# Autodesk Inventor assembly: 1000_Coil_Positioning_Assembly_MPSv2_v4
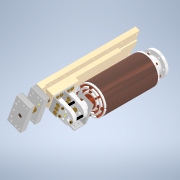
[picture p0: Inventor's stored thumbnail of the model, 180x180]
Saved by Autodesk Inventor 2021 (Build 250183000, 183)
## iProperties
Created: 2020-11-12
Part Number: 1000_Coil_Positioning_Assembly_MPSv2_v4
Document SubType Name: Assembly
Designer: Admin
Author: Admin
## Documents named in this file (23)
- C:\Users\Barksdale\Dropbox (MIT)\MPI Group Folder\MPS\MPSV2\1xxx Assemblies\1000_Coil_Positioning_Assembly_MPSv2_v4.iam
- C:\Users\Barksdale\Dropbox (MIT)\MPI Group Folder\MPS\MPSV2\2xxx Coil Formers and Parts\20xx Rx Coil\200x Rx Coil Solenoid Former\2000_Rx_Coil_Former_MPSv2_v2.ipt
- C:\Users\Barksdale\Dropbox (MIT)\MPI Group Folder\MPS\MPSV2\2xxx Coil Formers and Parts\20xx Rx Coil\200x Rx Coil Solenoid Former\2001_Fiberglass_Rod_MPSv2_v1.ipt
- C:\Users\Barksdale\Dropbox (MIT)\MPI Group Folder\MPS\MPSV2\2xxx Coil Formers and Parts\21xx Tx Coil\210x Tx Coil Solenoid Former\2100_Tx_Coil_Former_MPSv2_v3.ipt
- C:\Users\Barksdale\Dropbox (MIT)\MPI Group Folder\MPS\MPSV2\McMaster Carr Parts\94995A470_BRONZE THREADED ROD.ipt
- C:\Users\Barksdale\Dropbox (MIT)\MPI Group Folder\MPS\MPSV2\3xxx Coil Positioning and Support\30xx_Tx_Rx_Relative_Positioning\3004_Brass_Nut_0.25_20_Tx_Rx_Relative_Positioning_MPSv2_v1.ipt
- C:\Users\Barksdale\Dropbox (MIT)\MPI Group Folder\MPS\MPSV2\McMaster Carr Parts\98813A033_BRASS THREADED ROD.ipt
- C:\Users\Barksdale\Dropbox (MIT)\MPI Group Folder\MPS\MPSV2\3xxx Coil Positioning and Support\31xx_Bias_Coil_Positioning\311x_Bias_Tx_Rx_Relative_Positioning\3114_Brass_Nut_0.5_20_Tx_Rx_Relative_Positioning_MPSv2_v1.ipt
- C:\Users\Barksdale\Dropbox (MIT)\MPI Group Folder\MPS\MPSV2\McMaster Carr Parts\2705T140_LIGHT DUTY DRY-RUNNING FLANGED SLEEVE BEARING.ipt
- C:\Users\Barksdale\Dropbox (MIT)\MPI Group Folder\MPS\MPSV2\McMaster Carr Parts\2705T260_LIGHT DUTY DRY-RUNNING FLANGED SLEEVE BEARING.ipt
- C:\Users\Barksdale\Dropbox (MIT)\MPI Group Folder\MPS\MPSV2\3xxx Coil Positioning and Support\31xx_Bias_Coil_Positioning\311x_Bias_Tx_Rx_Relative_Positioning\3113_Bias_TxRx_Relative_Adapter_MPSv2_v1.ipt
- C:\Users\Barksdale\Dropbox (MIT)\MPI Group Folder\MPS\MPSV2\3xxx Coil Positioning and Support\31xx_Bias_Coil_Positioning\310x_Bias_Coil_Chasis_Mounting\3101_Bias_Coil_Mounting_Flange_MPSv2_v2.ipt
- C:\Users\Barksdale\Dropbox (MIT)\MPI Group Folder\MPS\MPSV2\2xxx Coil Formers and Parts\22xx Bias Coil\4000_Cu_Bias_Shielding_(McMaster_50475K18)_MPSv2_v2.ipt
- C:\Users\Barksdale\Dropbox (MIT)\MPI Group Folder\MPS\MPSV2\3xxx Coil Positioning and Support\30xx_Tx_Rx_Relative_Positioning\3000_Tx_Rx_Relative_Position_Adjust_Tx_Adadpter_Male_MPSv2_v5.ipt
- C:\Users\Barksdale\Dropbox (MIT)\MPI Group Folder\MPS\MPSV2\3xxx Coil Positioning and Support\31xx_Bias_Coil_Positioning\311x_Bias_Tx_Rx_Relative_Positioning\3112_Bias_TxRx_Relative_Dovetail_Male_MPSv2_v3.ipt
- C:\Users\Barksdale\Dropbox (MIT)\MPI Group Folder\MPS\MPSV2\3xxx Coil Positioning and Support\30xx_Tx_Rx_Relative_Positioning\3001_Tx_Rx_Relative_Position_Adjust_Tx_Adadpter_Female_MPSv2_v4.ipt
- C:\Users\Barksdale\Dropbox (MIT)\MPI Group Folder\MPS\MPSV2\3xxx Coil Positioning and Support\31xx_Bias_Coil_Positioning\311x_Bias_Tx_Rx_Relative_Positioning\3110_Bias_TxRx_Relative_Dovetail_Mount_Bracket_MPSv2_v4.ipt
- C:\Users\Barksdale\Dropbox (MIT)\MPI Group Folder\MPS\MPSV2\3xxx Coil Positioning and Support\31xx_Bias_Coil_Positioning\311x_Bias_Tx_Rx_Relative_Positioning\3111_Bias_TxRx_Relative_Dovetail_Female_MPSv2_v4.ipt
- C:\Users\Barksdale\Dropbox (MIT)\MPI Group Folder\MPS\MPSV2\3xxx Coil Positioning and Support\30xx_Tx_Rx_Relative_Positioning\3002_92451A838_BRASS FLAT HEAD SLOTTED MACHINE SCREW.ipt
- C:\Users\Barksdale\Dropbox (MIT)\MPI Group Folder\MPS\MPSV2\3xxx Coil Positioning and Support\30xx_Tx_Rx_Relative_Positioning\3003_95130A160_BRASS NARROW HEX NUT.ipt
- C:\Users\Barksdale\Dropbox (MIT)\MPI Group Folder\MPS\MPSV2\3xxx Coil Positioning and Support\31xx_Bias_Coil_Positioning\311x_Bias_Tx_Rx_Relative_Positioning\3115_94070A550_BRASS PAN HEAD PHILLIPS MACHINE SCREW.ipt
- C:\Users\Barksdale\Dropbox (MIT)\MPI Group Folder\MPS\MPSV2\1xxx Assemblies\10xx_Coil_Positioning_Assemblies\1002_Bias_Coil_MPSv2_v3.iam
- C:\Users\Barksdale\Dropbox (MIT)\MPI Group Folder\MPS\MPSV2\3xxx Coil Positioning and Support\31xx_Bias_Coil_Positioning\310x_Bias_Coil_Chasis_Mounting\3102_Biax_Coil_Mounting_Bracket_MPSv2_v1.ipt
## Components (46 placed, 22 different names)
1. 2000_Rx_Coil_Former_MPSv2_v2:1 — Mate:6, Mate:7, Mate:9, Angle:1, Flush:4
2. 2001_Fiberglass_Rod_MPSv2_v1:1 — Mate:6, Mate:7, Mate:20, Mate:124
3. 4000_Cu_Bias_Shielding_(McMaster_50475K18)_MPSv2_v2:1 — Mate:8, Mate:10, Mate:24, Mate:119, Mate:120, Mate:175, Mate:177, Mate:178
4. 2100_Tx_Coil_Former_MPSv2_v3:1 — Mate:8, Mate:9, Mate:10, Angle:1, Mate:25, Mate:26, Flush:4
5. 94995A470_BRONZE THREADED ROD:1 — Mate:20, Mate:81, Mate:124, Mate:128
6. 3004_Brass_Nut_0.25_20_Tx_Rx_Relative_Positioning_MPSv2_v1:1 — Mate:74, Mate:75, Mate:76, Mate:77
7. 3000_Tx_Rx_Relative_Position_Adjust_Tx_Adadpter_Male_MPSv2_v5:1 — Mate:24, Mate:25, Mate:26, Mate:129, Mate:133
8. 3110_Bias_TxRx_Relative_Dovetail_Mount_Bracket_MPSv2_v4:2 — Mate:83, Mate:130, Mate:131, Mate:141, Mate:142, Mate:155, Mate:157, Mate:160, Mate:161, Mate:166, Mate:167, Mate:168, Mate:169, Mate:174
9. 3110_Bias_TxRx_Relative_Dovetail_Mount_Bracket_MPSv2_v4:1 — Mate:56, Mate:137, Mate:139, Mate:140, Mate:154, Mate:165, Mate:170, Mate:171, Mate:172, Mate:173
10. 3111_Bias_TxRx_Relative_Dovetail_Female_MPSv2_v4:1 — Mate:56, Mate:59, Mate:62, Mate:63, Mate:83, Mate:141, Mate:142, Mate:144
11. 98813A033_BRASS THREADED ROD:1 — Mate:59, Mate:64, Mate:65, Mate:144
12. 3112_Bias_TxRx_Relative_Dovetail_Male_MPSv2_v3:1 — Mate:62, Mate:63, Mate:99, Mate:100, Mate:125, Angle:2
13. 98813A033_BRASS THREADED ROD:2 — Mate:64, Mate:65, Mate:91
14. 3114_Brass_Nut_0.5_20_Tx_Rx_Relative_Positioning_MPSv2_v1:1 — Mate:87, Mate:88, Mate:89, Mate:90
15. 2705T140_LIGHT DUTY DRY-RUNNING FLANGED SLEEVE BEARING:1 — Mate:74, Mate:75, Mate:135, Mate:136
16. 2705T140_LIGHT DUTY DRY-RUNNING FLANGED SLEEVE BEARING:2 — Mate:76, Mate:77, Mate:81, Mate:134
17. 2705T260_LIGHT DUTY DRY-RUNNING FLANGED SLEEVE BEARING:1 — Mate:87, Mate:90, Mate:91, Mate:102
18. 2705T260_LIGHT DUTY DRY-RUNNING FLANGED SLEEVE BEARING:2 — Mate:88, Mate:89, Mate:98, Mate:103
19. 3113_Bias_TxRx_Relative_Adapter_MPSv2_v1:1 — Mate:99, Mate:100, Mate:102, Mate:104, Mate:105, Mate:125
20. 3113_Bias_TxRx_Relative_Adapter_MPSv2_v1:2 — Mate:98, Mate:103, Mate:104, Mate:105
21. 3101_Bias_Coil_Mounting_Flange_MPSv2_v2:1 — Mate:119, Mate:120, Mate:176
22. 1002_Bias_Coil_MPSv2_v3:1 [sub-assembly] — Mate:175, Mate:176
23. 3001_Tx_Rx_Relative_Position_Adjust_Tx_Adadpter_Female_MPSv2_v4:1 — Mate:128, Mate:129, Mate:130, Mate:131, Mate:133, Mate:134, Flush:6, Mate:145, Mate:146, Mate:147, Flush:7, Flush:8, Flush:9, Mate:155, Mate:156, Mate:158, Mate:159
24. 3001_Tx_Rx_Relative_Position_Adjust_Tx_Adadpter_Female_MPSv2_v4:2 — Mate:135, Flush:6, Mate:136, Mate:137, Mate:139, Mate:140, Mate:148, Mate:149, Mate:150, Mate:154, Mate:162, Mate:163, Mate:164
25. 3002_92451A838_BRASS FLAT HEAD SLOTTED MACHINE SCREW:1 — Mate:145, Flush:7, Mate:151
26. 3002_92451A838_BRASS FLAT HEAD SLOTTED MACHINE SCREW:2 — Mate:147, Flush:8, Mate:153
27. 3002_92451A838_BRASS FLAT HEAD SLOTTED MACHINE SCREW:3 — Mate:146, Flush:9, Mate:152
28. 3003_95130A160_BRASS NARROW HEX NUT:1 — Mate:150, Mate:152
29. 3003_95130A160_BRASS NARROW HEX NUT:2 — Mate:148, Mate:153
30. 3003_95130A160_BRASS NARROW HEX NUT:3 — Mate:149, Mate:151
31. 3115_94070A550_BRASS PAN HEAD PHILLIPS MACHINE SCREW:1 — Mate:156, Mate:157
32. 3115_94070A550_BRASS PAN HEAD PHILLIPS MACHINE SCREW:2 — Mate:159, Mate:160
33. 3115_94070A550_BRASS PAN HEAD PHILLIPS MACHINE SCREW:3 — Mate:158, Mate:161
34. 3115_94070A550_BRASS PAN HEAD PHILLIPS MACHINE SCREW:4 — Flush:10, Flush:11, Mate:162, Mate:165
35. 3115_94070A550_BRASS PAN HEAD PHILLIPS MACHINE SCREW:5 — Flush:10, Mate:163
36. 3115_94070A550_BRASS PAN HEAD PHILLIPS MACHINE SCREW:6 — Flush:11, Mate:164
37. 3115_94070A550_BRASS PAN HEAD PHILLIPS MACHINE SCREW:7 — Flush:18, Mate:166, Mate:174
38. 3115_94070A550_BRASS PAN HEAD PHILLIPS MACHINE SCREW:8 — Flush:16, Mate:168
39. 3115_94070A550_BRASS PAN HEAD PHILLIPS MACHINE SCREW:9 — Flush:17, Mate:167
40. 3115_94070A550_BRASS PAN HEAD PHILLIPS MACHINE SCREW:10 — Flush:15, Mate:169
41. 3115_94070A550_BRASS PAN HEAD PHILLIPS MACHINE SCREW:11 — Flush:12, Flush:14, Flush:15, Flush:16, Flush:17, Flush:18, Mate:170
42. 3115_94070A550_BRASS PAN HEAD PHILLIPS MACHINE SCREW:12 — Flush:12, Flush:13, Mate:172
43. 3115_94070A550_BRASS PAN HEAD PHILLIPS MACHINE SCREW:13 — Flush:13, Mate:173
44. 3115_94070A550_BRASS PAN HEAD PHILLIPS MACHINE SCREW:14 — Flush:14, Mate:171
45. 3102_Biax_Coil_Mounting_Bracket_MPSv2_v1:1 — Mate:177, Mate:178, Mate:179, Flush:19, Flush:20
46. 3110_Bias_TxRx_Relative_Dovetail_Mount_Bracket_MPSv2_v4:3 — Mate:179, Flush:19, Angle:2, Flush:20
## Relationships (104: Mate 86, Flush 16, Angle 2)
- Mate:6: 2000_Rx_Coil_Former_MPSv2_v2:1 ↔ 2001_Fiberglass_Rod_MPSv2_v1:1
- Mate:7: 2000_Rx_Coil_Former_MPSv2_v2:1 ↔ 2001_Fiberglass_Rod_MPSv2_v1:1
- Mate:8: 4000_Cu_Bias_Shielding_(McMaster_50475K18)_MPSv2_v2:1 ↔ 2100_Tx_Coil_Former_MPSv2_v3:1
- Mate:9: 2000_Rx_Coil_Former_MPSv2_v2:1 ↔ 2100_Tx_Coil_Former_MPSv2_v3:1
- Mate:10: 4000_Cu_Bias_Shielding_(McMaster_50475K18)_MPSv2_v2:1 ↔ 2100_Tx_Coil_Former_MPSv2_v3:1
- Angle:1 (0 deg): 2000_Rx_Coil_Former_MPSv2_v2:1 ↔ 2100_Tx_Coil_Former_MPSv2_v3:1
- Mate:20: 2001_Fiberglass_Rod_MPSv2_v1:1 ↔ 94995A470_BRONZE THREADED ROD:1
- Mate:24: 4000_Cu_Bias_Shielding_(McMaster_50475K18)_MPSv2_v2:1 ↔ 3000_Tx_Rx_Relative_Position_Adjust_Tx_Adadpter_Male_MPSv2_v5:1
- Mate:25: 2100_Tx_Coil_Former_MPSv2_v3:1 ↔ 3000_Tx_Rx_Relative_Position_Adjust_Tx_Adadpter_Male_MPSv2_v5:1
- Mate:26: 2100_Tx_Coil_Former_MPSv2_v3:1 ↔ 3000_Tx_Rx_Relative_Position_Adjust_Tx_Adadpter_Male_MPSv2_v5:1
- Mate:56: 3110_Bias_TxRx_Relative_Dovetail_Mount_Bracket_MPSv2_v4:1 ↔ 3111_Bias_TxRx_Relative_Dovetail_Female_MPSv2_v4:1
- Mate:59: 3111_Bias_TxRx_Relative_Dovetail_Female_MPSv2_v4:1 ↔ 98813A033_BRASS THREADED ROD:1
- Mate:62: 3111_Bias_TxRx_Relative_Dovetail_Female_MPSv2_v4:1 ↔ 3112_Bias_TxRx_Relative_Dovetail_Male_MPSv2_v3:1
- Mate:63: 3111_Bias_TxRx_Relative_Dovetail_Female_MPSv2_v4:1 ↔ 3112_Bias_TxRx_Relative_Dovetail_Male_MPSv2_v3:1
- Mate:64: 98813A033_BRASS THREADED ROD:1 ↔ 98813A033_BRASS THREADED ROD:2
- Mate:65 (-5 mm): 98813A033_BRASS THREADED ROD:1 ↔ 98813A033_BRASS THREADED ROD:2
- Mate:74: 3004_Brass_Nut_0.25_20_Tx_Rx_Relative_Positioning_MPSv2_v1:1 ↔ 2705T140_LIGHT DUTY DRY-RUNNING FLANGED SLEEVE BEARING:1
- Mate:75: 3004_Brass_Nut_0.25_20_Tx_Rx_Relative_Positioning_MPSv2_v1:1 ↔ 2705T140_LIGHT DUTY DRY-RUNNING FLANGED SLEEVE BEARING:1
- Mate:76: 3004_Brass_Nut_0.25_20_Tx_Rx_Relative_Positioning_MPSv2_v1:1 ↔ 2705T140_LIGHT DUTY DRY-RUNNING FLANGED SLEEVE BEARING:2
- Mate:77: 3004_Brass_Nut_0.25_20_Tx_Rx_Relative_Positioning_MPSv2_v1:1 ↔ 2705T140_LIGHT DUTY DRY-RUNNING FLANGED SLEEVE BEARING:2
- Mate:81: 94995A470_BRONZE THREADED ROD:1 ↔ 2705T140_LIGHT DUTY DRY-RUNNING FLANGED SLEEVE BEARING:2
- Mate:83: 3110_Bias_TxRx_Relative_Dovetail_Mount_Bracket_MPSv2_v4:2 ↔ 3111_Bias_TxRx_Relative_Dovetail_Female_MPSv2_v4:1
- Mate:87: 3114_Brass_Nut_0.5_20_Tx_Rx_Relative_Positioning_MPSv2_v1:1 ↔ 2705T260_LIGHT DUTY DRY-RUNNING FLANGED SLEEVE BEARING:1
- Mate:88: 3114_Brass_Nut_0.5_20_Tx_Rx_Relative_Positioning_MPSv2_v1:1 ↔ 2705T260_LIGHT DUTY DRY-RUNNING FLANGED SLEEVE BEARING:2
- Mate:89: 3114_Brass_Nut_0.5_20_Tx_Rx_Relative_Positioning_MPSv2_v1:1 ↔ 2705T260_LIGHT DUTY DRY-RUNNING FLANGED SLEEVE BEARING:2
- Mate:90: 3114_Brass_Nut_0.5_20_Tx_Rx_Relative_Positioning_MPSv2_v1:1 ↔ 2705T260_LIGHT DUTY DRY-RUNNING FLANGED SLEEVE BEARING:1
- Mate:91: 98813A033_BRASS THREADED ROD:2 ↔ 2705T260_LIGHT DUTY DRY-RUNNING FLANGED SLEEVE BEARING:1
- Mate:98: 2705T260_LIGHT DUTY DRY-RUNNING FLANGED SLEEVE BEARING:2 ↔ 3113_Bias_TxRx_Relative_Adapter_MPSv2_v1:2
- Mate:99: 3112_Bias_TxRx_Relative_Dovetail_Male_MPSv2_v3:1 ↔ 3113_Bias_TxRx_Relative_Adapter_MPSv2_v1:1
- Mate:100: 3112_Bias_TxRx_Relative_Dovetail_Male_MPSv2_v3:1 ↔ 3113_Bias_TxRx_Relative_Adapter_MPSv2_v1:1
- Mate:102: 2705T260_LIGHT DUTY DRY-RUNNING FLANGED SLEEVE BEARING:1 ↔ 3113_Bias_TxRx_Relative_Adapter_MPSv2_v1:1
- Mate:103: 2705T260_LIGHT DUTY DRY-RUNNING FLANGED SLEEVE BEARING:2 ↔ 3113_Bias_TxRx_Relative_Adapter_MPSv2_v1:2
- Mate:104: 3113_Bias_TxRx_Relative_Adapter_MPSv2_v1:1 ↔ 3113_Bias_TxRx_Relative_Adapter_MPSv2_v1:2
- Mate:105: 3113_Bias_TxRx_Relative_Adapter_MPSv2_v1:1 ↔ 3113_Bias_TxRx_Relative_Adapter_MPSv2_v1:2
- Flush:4: 2000_Rx_Coil_Former_MPSv2_v2:1 ↔ 2100_Tx_Coil_Former_MPSv2_v3:1
- Mate:119: 4000_Cu_Bias_Shielding_(McMaster_50475K18)_MPSv2_v2:1 ↔ 3101_Bias_Coil_Mounting_Flange_MPSv2_v2:1
- Mate:120: 4000_Cu_Bias_Shielding_(McMaster_50475K18)_MPSv2_v2:1 ↔ 3101_Bias_Coil_Mounting_Flange_MPSv2_v2:1
- Mate:124: 2001_Fiberglass_Rod_MPSv2_v1:1 ↔ 94995A470_BRONZE THREADED ROD:1
- Mate:125: 3112_Bias_TxRx_Relative_Dovetail_Male_MPSv2_v3:1 ↔ 3113_Bias_TxRx_Relative_Adapter_MPSv2_v1:1
- Mate:128: 94995A470_BRONZE THREADED ROD:1 ↔ 3001_Tx_Rx_Relative_Position_Adjust_Tx_Adadpter_Female_MPSv2_v4:1
- Mate:129: 3000_Tx_Rx_Relative_Position_Adjust_Tx_Adadpter_Male_MPSv2_v5:1 ↔ 3001_Tx_Rx_Relative_Position_Adjust_Tx_Adadpter_Female_MPSv2_v4:1
- Mate:130: 3110_Bias_TxRx_Relative_Dovetail_Mount_Bracket_MPSv2_v4:2 ↔ 3001_Tx_Rx_Relative_Position_Adjust_Tx_Adadpter_Female_MPSv2_v4:1
- Mate:131: 3110_Bias_TxRx_Relative_Dovetail_Mount_Bracket_MPSv2_v4:2 ↔ 3001_Tx_Rx_Relative_Position_Adjust_Tx_Adadpter_Female_MPSv2_v4:1
- Mate:133: 3000_Tx_Rx_Relative_Position_Adjust_Tx_Adadpter_Male_MPSv2_v5:1 ↔ 3001_Tx_Rx_Relative_Position_Adjust_Tx_Adadpter_Female_MPSv2_v4:1
- Mate:134: 2705T140_LIGHT DUTY DRY-RUNNING FLANGED SLEEVE BEARING:2 ↔ 3001_Tx_Rx_Relative_Position_Adjust_Tx_Adadpter_Female_MPSv2_v4:1
- Mate:135: 2705T140_LIGHT DUTY DRY-RUNNING FLANGED SLEEVE BEARING:1 ↔ 3001_Tx_Rx_Relative_Position_Adjust_Tx_Adadpter_Female_MPSv2_v4:2
- Flush:6: 3001_Tx_Rx_Relative_Position_Adjust_Tx_Adadpter_Female_MPSv2_v4:1 ↔ 3001_Tx_Rx_Relative_Position_Adjust_Tx_Adadpter_Female_MPSv2_v4:2
- Mate:136: 2705T140_LIGHT DUTY DRY-RUNNING FLANGED SLEEVE BEARING:1 ↔ 3001_Tx_Rx_Relative_Position_Adjust_Tx_Adadpter_Female_MPSv2_v4:2
- Mate:137: 3110_Bias_TxRx_Relative_Dovetail_Mount_Bracket_MPSv2_v4:1 ↔ 3001_Tx_Rx_Relative_Position_Adjust_Tx_Adadpter_Female_MPSv2_v4:2
- Mate:139: 3110_Bias_TxRx_Relative_Dovetail_Mount_Bracket_MPSv2_v4:1 ↔ 3001_Tx_Rx_Relative_Position_Adjust_Tx_Adadpter_Female_MPSv2_v4:2
- Mate:140: 3110_Bias_TxRx_Relative_Dovetail_Mount_Bracket_MPSv2_v4:1 ↔ 3001_Tx_Rx_Relative_Position_Adjust_Tx_Adadpter_Female_MPSv2_v4:2
- Mate:141: 3110_Bias_TxRx_Relative_Dovetail_Mount_Bracket_MPSv2_v4:2 ↔ 3111_Bias_TxRx_Relative_Dovetail_Female_MPSv2_v4:1
- Mate:142: 3110_Bias_TxRx_Relative_Dovetail_Mount_Bracket_MPSv2_v4:2 ↔ 3111_Bias_TxRx_Relative_Dovetail_Female_MPSv2_v4:1
- Mate:144: 3111_Bias_TxRx_Relative_Dovetail_Female_MPSv2_v4:1 ↔ 98813A033_BRASS THREADED ROD:1
- Mate:145: 3001_Tx_Rx_Relative_Position_Adjust_Tx_Adadpter_Female_MPSv2_v4:1 ↔ 3002_92451A838_BRASS FLAT HEAD SLOTTED MACHINE SCREW:1
- Mate:146: 3001_Tx_Rx_Relative_Position_Adjust_Tx_Adadpter_Female_MPSv2_v4:1 ↔ 3002_92451A838_BRASS FLAT HEAD SLOTTED MACHINE SCREW:3
- Mate:147: 3001_Tx_Rx_Relative_Position_Adjust_Tx_Adadpter_Female_MPSv2_v4:1 ↔ 3002_92451A838_BRASS FLAT HEAD SLOTTED MACHINE SCREW:2
- Flush:7: 3001_Tx_Rx_Relative_Position_Adjust_Tx_Adadpter_Female_MPSv2_v4:1 ↔ 3002_92451A838_BRASS FLAT HEAD SLOTTED MACHINE SCREW:1
- Flush:8: 3001_Tx_Rx_Relative_Position_Adjust_Tx_Adadpter_Female_MPSv2_v4:1 ↔ 3002_92451A838_BRASS FLAT HEAD SLOTTED MACHINE SCREW:2
- Flush:9: 3001_Tx_Rx_Relative_Position_Adjust_Tx_Adadpter_Female_MPSv2_v4:1 ↔ 3002_92451A838_BRASS FLAT HEAD SLOTTED MACHINE SCREW:3
- Mate:148: 3001_Tx_Rx_Relative_Position_Adjust_Tx_Adadpter_Female_MPSv2_v4:2 ↔ 3003_95130A160_BRASS NARROW HEX NUT:2
- Mate:149: 3001_Tx_Rx_Relative_Position_Adjust_Tx_Adadpter_Female_MPSv2_v4:2 ↔ 3003_95130A160_BRASS NARROW HEX NUT:3
- Mate:150: 3001_Tx_Rx_Relative_Position_Adjust_Tx_Adadpter_Female_MPSv2_v4:2 ↔ 3003_95130A160_BRASS NARROW HEX NUT:1
- Mate:151: 3002_92451A838_BRASS FLAT HEAD SLOTTED MACHINE SCREW:1 ↔ 3003_95130A160_BRASS NARROW HEX NUT:3
- Mate:152: 3002_92451A838_BRASS FLAT HEAD SLOTTED MACHINE SCREW:3 ↔ 3003_95130A160_BRASS NARROW HEX NUT:1
- Mate:153: 3002_92451A838_BRASS FLAT HEAD SLOTTED MACHINE SCREW:2 ↔ 3003_95130A160_BRASS NARROW HEX NUT:2
- Mate:154: 3110_Bias_TxRx_Relative_Dovetail_Mount_Bracket_MPSv2_v4:1 ↔ 3001_Tx_Rx_Relative_Position_Adjust_Tx_Adadpter_Female_MPSv2_v4:2
- Mate:155: 3110_Bias_TxRx_Relative_Dovetail_Mount_Bracket_MPSv2_v4:2 ↔ 3001_Tx_Rx_Relative_Position_Adjust_Tx_Adadpter_Female_MPSv2_v4:1
- Mate:156: 3001_Tx_Rx_Relative_Position_Adjust_Tx_Adadpter_Female_MPSv2_v4:1 ↔ 3115_94070A550_BRASS PAN HEAD PHILLIPS MACHINE SCREW:1
- Mate:157: 3110_Bias_TxRx_Relative_Dovetail_Mount_Bracket_MPSv2_v4:2 ↔ 3115_94070A550_BRASS PAN HEAD PHILLIPS MACHINE SCREW:1
- Mate:158: 3001_Tx_Rx_Relative_Position_Adjust_Tx_Adadpter_Female_MPSv2_v4:1 ↔ 3115_94070A550_BRASS PAN HEAD PHILLIPS MACHINE SCREW:3
- Mate:159: 3001_Tx_Rx_Relative_Position_Adjust_Tx_Adadpter_Female_MPSv2_v4:1 ↔ 3115_94070A550_BRASS PAN HEAD PHILLIPS MACHINE SCREW:2
- Mate:160: 3110_Bias_TxRx_Relative_Dovetail_Mount_Bracket_MPSv2_v4:2 ↔ 3115_94070A550_BRASS PAN HEAD PHILLIPS MACHINE SCREW:2
- Mate:161: 3110_Bias_TxRx_Relative_Dovetail_Mount_Bracket_MPSv2_v4:2 ↔ 3115_94070A550_BRASS PAN HEAD PHILLIPS MACHINE SCREW:3
- Flush:10: 3115_94070A550_BRASS PAN HEAD PHILLIPS MACHINE SCREW:4 ↔ 3115_94070A550_BRASS PAN HEAD PHILLIPS MACHINE SCREW:5
- Flush:11: 3115_94070A550_BRASS PAN HEAD PHILLIPS MACHINE SCREW:4 ↔ 3115_94070A550_BRASS PAN HEAD PHILLIPS MACHINE SCREW:6
- Mate:162: 3001_Tx_Rx_Relative_Position_Adjust_Tx_Adadpter_Female_MPSv2_v4:2 ↔ 3115_94070A550_BRASS PAN HEAD PHILLIPS MACHINE SCREW:4
- Mate:163: 3001_Tx_Rx_Relative_Position_Adjust_Tx_Adadpter_Female_MPSv2_v4:2 ↔ 3115_94070A550_BRASS PAN HEAD PHILLIPS MACHINE SCREW:5
- Mate:164: 3001_Tx_Rx_Relative_Position_Adjust_Tx_Adadpter_Female_MPSv2_v4:2 ↔ 3115_94070A550_BRASS PAN HEAD PHILLIPS MACHINE SCREW:6
- Mate:165: 3110_Bias_TxRx_Relative_Dovetail_Mount_Bracket_MPSv2_v4:1 ↔ 3115_94070A550_BRASS PAN HEAD PHILLIPS MACHINE SCREW:4
- Flush:12: 3115_94070A550_BRASS PAN HEAD PHILLIPS MACHINE SCREW:11 ↔ 3115_94070A550_BRASS PAN HEAD PHILLIPS MACHINE SCREW:12
- Flush:13: 3115_94070A550_BRASS PAN HEAD PHILLIPS MACHINE SCREW:12 ↔ 3115_94070A550_BRASS PAN HEAD PHILLIPS MACHINE SCREW:13
- Flush:14: 3115_94070A550_BRASS PAN HEAD PHILLIPS MACHINE SCREW:11 ↔ 3115_94070A550_BRASS PAN HEAD PHILLIPS MACHINE SCREW:14
- Flush:15: 3115_94070A550_BRASS PAN HEAD PHILLIPS MACHINE SCREW:10 ↔ 3115_94070A550_BRASS PAN HEAD PHILLIPS MACHINE SCREW:11
- Flush:16: 3115_94070A550_BRASS PAN HEAD PHILLIPS MACHINE SCREW:8 ↔ 3115_94070A550_BRASS PAN HEAD PHILLIPS MACHINE SCREW:11
- Flush:17: 3115_94070A550_BRASS PAN HEAD PHILLIPS MACHINE SCREW:9 ↔ 3115_94070A550_BRASS PAN HEAD PHILLIPS MACHINE SCREW:11
- Flush:18: 3115_94070A550_BRASS PAN HEAD PHILLIPS MACHINE SCREW:7 ↔ 3115_94070A550_BRASS PAN HEAD PHILLIPS MACHINE SCREW:11
- Mate:166: 3110_Bias_TxRx_Relative_Dovetail_Mount_Bracket_MPSv2_v4:2 ↔ 3115_94070A550_BRASS PAN HEAD PHILLIPS MACHINE SCREW:7
- Mate:167: 3110_Bias_TxRx_Relative_Dovetail_Mount_Bracket_MPSv2_v4:2 ↔ 3115_94070A550_BRASS PAN HEAD PHILLIPS MACHINE SCREW:9
- Mate:168: 3110_Bias_TxRx_Relative_Dovetail_Mount_Bracket_MPSv2_v4:2 ↔ 3115_94070A550_BRASS PAN HEAD PHILLIPS MACHINE SCREW:8
- Mate:169: 3110_Bias_TxRx_Relative_Dovetail_Mount_Bracket_MPSv2_v4:2 ↔ 3115_94070A550_BRASS PAN HEAD PHILLIPS MACHINE SCREW:10
- Mate:170: 3110_Bias_TxRx_Relative_Dovetail_Mount_Bracket_MPSv2_v4:1 ↔ 3115_94070A550_BRASS PAN HEAD PHILLIPS MACHINE SCREW:11
- Mate:171: 3110_Bias_TxRx_Relative_Dovetail_Mount_Bracket_MPSv2_v4:1 ↔ 3115_94070A550_BRASS PAN HEAD PHILLIPS MACHINE SCREW:14
- Mate:172: 3110_Bias_TxRx_Relative_Dovetail_Mount_Bracket_MPSv2_v4:1 ↔ 3115_94070A550_BRASS PAN HEAD PHILLIPS MACHINE SCREW:12
- Mate:173: 3110_Bias_TxRx_Relative_Dovetail_Mount_Bracket_MPSv2_v4:1 ↔ 3115_94070A550_BRASS PAN HEAD PHILLIPS MACHINE SCREW:13
- Mate:174: 3110_Bias_TxRx_Relative_Dovetail_Mount_Bracket_MPSv2_v4:2 ↔ 3115_94070A550_BRASS PAN HEAD PHILLIPS MACHINE SCREW:7
- Mate:175: 4000_Cu_Bias_Shielding_(McMaster_50475K18)_MPSv2_v2:1 ↔ 1002_Bias_Coil_MPSv2_v3:1
- Mate:176: 3101_Bias_Coil_Mounting_Flange_MPSv2_v2:1 ↔ 1002_Bias_Coil_MPSv2_v3:1
- Mate:177: 4000_Cu_Bias_Shielding_(McMaster_50475K18)_MPSv2_v2:1 ↔ 3102_Biax_Coil_Mounting_Bracket_MPSv2_v1:1
- Mate:178: 4000_Cu_Bias_Shielding_(McMaster_50475K18)_MPSv2_v2:1 ↔ 3102_Biax_Coil_Mounting_Bracket_MPSv2_v1:1
- Mate:179: 3102_Biax_Coil_Mounting_Bracket_MPSv2_v1:1 ↔ 3110_Bias_TxRx_Relative_Dovetail_Mount_Bracket_MPSv2_v4:3
- Flush:19: 3102_Biax_Coil_Mounting_Bracket_MPSv2_v1:1 ↔ 3110_Bias_TxRx_Relative_Dovetail_Mount_Bracket_MPSv2_v4:3
- Angle:2 (0 deg): 3112_Bias_TxRx_Relative_Dovetail_Male_MPSv2_v3:1 ↔ 3110_Bias_TxRx_Relative_Dovetail_Mount_Bracket_MPSv2_v4:3
- Flush:20: 3102_Biax_Coil_Mounting_Bracket_MPSv2_v1:1 ↔ 3110_Bias_TxRx_Relative_Dovetail_Mount_Bracket_MPSv2_v4:3
